# Autodesk Inventor assembly: Gantry Assembly
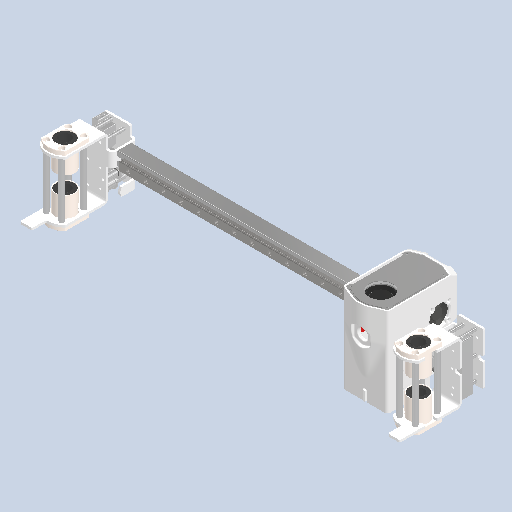
[picture p0: Inventor's stored thumbnail of the model, 512x512]
Saved by Autodesk Inventor 2024 (Build 280153000, 153)
## iProperties
Created: 2024-12-26
Part Number: Gantry Assembly
Document SubType Name: Assembly
Designer: Ishaan
Author: Ishaan
## Documents named in this file (15)
- E:\Projects\Axiom--IDEX-3D-Printer\CAD\04 - Gantry\Gantry Assembly.iam
- E:\Projects\Axiom--IDEX-3D-Printer\CAD\04 - Gantry\Left Gantry Guide.ipt
- E:\Projects\Axiom--IDEX-3D-Printer\CAD\00 - COTS Components\LMH16UU\LMH16UUx37\LMH16UUx37.ipt
- E:\Projects\Axiom--IDEX-3D-Printer\CAD\00 - COTS Components\Hardware\M3 30mm Standoff.ipt
- E:\Projects\Axiom--IDEX-3D-Printer\CAD\04 - Gantry\Right Gantry Guide.ipt
- E:\Projects\Axiom--IDEX-3D-Printer\CAD\04 - Gantry\Gantry Belt Clamp.ipt
- E:\Projects\Axiom--IDEX-3D-Printer\CAD\04 - Gantry\Gantry Belt Retainer.ipt
- E:\Projects\Axiom--IDEX-3D-Printer\CAD\00 - COTS Components\10mm 20T GT2 Idler Pulley 5mm Bore\10mm 20T GT2 Idler Pulley 5mm Bore.ipt
- E:\Projects\Axiom--IDEX-3D-Printer\CAD\00 - COTS Components\10mm Smooth Idler Pulley 5mm Bore\10mm 20T Smooth Idler Pulley 5mm Bore.ipt
- E:\Projects\Axiom--IDEX-3D-Printer\CAD\00 - COTS Components\Hardware\M5 Shim 0p5mm.ipt
- E:\Projects\Axiom--IDEX-3D-Printer\CAD\00 - COTS Components\Hardware\M5 Spacer 15mm.ipt
- E:\Projects\Axiom--IDEX-3D-Printer\CAD\00 - COTS Components\MGNR12 Rail\MGNR12R475HM.ipt
- E:\Projects\Axiom--IDEX-3D-Printer\CAD\05 - Printhead\Printhead Assembly.iam
- E:\Projects\Axiom--IDEX-3D-Printer\CAD\00 - COTS Components\Hardware\M4 80mm Standoff.ipt
- E:\Projects\Axiom--IDEX-3D-Printer\CAD\00 - COTS Components\2020 Gantry Extrusion\HFSH5-2020-446.ipt
## Components (57 placed, 14 different names)
1. Left Gantry Guide:1 — Insert:1, Insert:2, Insert:3, Insert:4, Insert:9, Insert:10, Insert:11, Insert:12, Insert:13, Insert:14, Insert:15, Insert:34, Insert:35, Insert:56, Insert:57, Insert:58, Insert:65, Insert:66, Insert:67
2. Right Gantry Guide:1 — Insert:17, Insert:18, Insert:19, Insert:20, Insert:25, Insert:26, Insert:27, Insert:28, Insert:29, Insert:30, Insert:31, Insert:48, Insert:49, Insert:52, Insert:54, Insert:62, Insert:63, Insert:64
3. HFSH5-2020-446:1
4. LMH16UUx37:1 — Insert:1, Insert:2
5. LMH16UUx37:2 — Insert:3, Insert:4
6. LMH16UUx37:3 — Insert:19, Insert:20
7. LMH16UUx37:4 — Insert:17, Insert:18
8. Gantry Belt Clamp:1 — Insert:36, Insert:37, Insert:38, Insert:39
9. Gantry Belt Retainer:1 — Insert:40, Insert:41
10. Gantry Belt Clamp:2 — Insert:38, Insert:39, Insert:40, Insert:41
11. Gantry Belt Retainer:2 — Insert:34, Insert:35, Insert:36, Insert:37
12. Gantry Belt Clamp:3
13. Gantry Belt Retainer:3
14. Gantry Belt Clamp:4
15. Gantry Belt Retainer:4 — Insert:48, Insert:49
16. 10mm 20T GT2 Idler Pulley 5mm Bore:1 — Insert:55
17. 10mm 20T GT2 Idler Pulley 5mm Bore:2 — Insert:61
18. 10mm 20T Smooth Idler Pulley 5mm Bore:1 — Insert:60
19. 10mm 20T Smooth Idler Pulley 5mm Bore:2 — Insert:59
20. 10mm 20T Smooth Idler Pulley 5mm Bore:3 — Insert:51
21. 10mm 20T Smooth Idler Pulley 5mm Bore:4 — Insert:53
22. M5 Spacer 15mm:1 — Insert:64
23. M5 Spacer 15mm:2 — Insert:63
24. M5 Spacer 15mm:3 — Insert:62
25. M5 Spacer 15mm:4 — Insert:67
26. M5 Spacer 15mm:5 — Insert:66
27. M5 Spacer 15mm:6 — Insert:65
28. MGNR12R475HM:1 — Mate:5
29. Printhead Assembly:1 [sub-assembly] — Mate:5
30. M5 Shim 0p5mm:1 — Insert:50, Insert:51
31. M5 Shim 0p5mm:2 — Insert:54, Insert:55
32. M5 Shim 0p5mm:3 — Insert:52, Insert:53
33. M5 Shim 0p5mm:4 — Insert:58, Insert:59
34. M5 Shim 0p5mm:5 — Insert:56, Insert:60
35. M5 Shim 0p5mm:6 — Insert:57, Insert:61
36. M3 30mm Standoff:8 — Insert:25
37. M3 30mm Standoff:9 — Insert:27
38. M3 30mm Standoff:10 — Insert:26
39. M3 30mm Standoff:11 — Insert:29
40. M3 30mm Standoff:12 — Insert:30
41. M3 30mm Standoff:13 — Insert:31
42. M3 30mm Standoff:14 — Insert:28, Insert:50
43. M4 80mm Standoff:1
44. M4 80mm Standoff:2
45. M4 80mm Standoff:3
46. M4 80mm Standoff:4
47. M4 80mm Standoff:5
48. M4 80mm Standoff:6
49. M4 80mm Standoff:7
50. M4 80mm Standoff:8
51. M3 30mm Standoff:1 — Insert:10
52. M3 30mm Standoff:2 — Insert:11
53. M3 30mm Standoff:3 — Insert:12
54. M3 30mm Standoff:4 — Insert:13
55. M3 30mm Standoff:5 — Insert:14
56. M3 30mm Standoff:6 — Insert:15
57. M3 30mm Standoff:7 — Insert:9
## Relationships (73: Insert 66, Mate 5, Angle 2)
- Insert:1: Left Gantry Guide:1 ↔ LMH16UUx37:1
- Insert:2: Left Gantry Guide:1 ↔ LMH16UUx37:1
- Insert:3: Left Gantry Guide:1 ↔ LMH16UUx37:2
- Insert:4: Left Gantry Guide:1 ↔ LMH16UUx37:2
- [Insert]: Left Gantry Guide:1 ↔ M4 80mm Standoff:8
- [Insert]: Left Gantry Guide:1 ↔ M4 80mm Standoff:7
- [Insert]: Left Gantry Guide:1 ↔ M4 80mm Standoff:6
- [Insert]: Left Gantry Guide:1 ↔ M4 80mm Standoff:5
- Insert:9: Left Gantry Guide:1 ↔ M3 30mm Standoff:7
- Insert:10: Left Gantry Guide:1 ↔ M3 30mm Standoff:1
- Insert:11: Left Gantry Guide:1 ↔ M3 30mm Standoff:2
- Insert:12: Left Gantry Guide:1 ↔ M3 30mm Standoff:3
- Insert:13: Left Gantry Guide:1 ↔ M3 30mm Standoff:4
- Insert:14: Left Gantry Guide:1 ↔ M3 30mm Standoff:5
- Insert:15: Left Gantry Guide:1 ↔ M3 30mm Standoff:6
- Insert:17: Right Gantry Guide:1 ↔ LMH16UUx37:4
- Insert:18: Right Gantry Guide:1 ↔ LMH16UUx37:4
- Insert:19: Right Gantry Guide:1 ↔ LMH16UUx37:3
- Insert:20: Right Gantry Guide:1 ↔ LMH16UUx37:3
- [Insert]: Right Gantry Guide:1 ↔ M4 80mm Standoff:1
- [Insert]: Right Gantry Guide:1 ↔ M4 80mm Standoff:2
- [Insert]: Right Gantry Guide:1 ↔ M4 80mm Standoff:3
- [Insert]: Right Gantry Guide:1 ↔ M4 80mm Standoff:4
- Insert:25: Right Gantry Guide:1 ↔ M3 30mm Standoff:8
- Insert:26: Right Gantry Guide:1 ↔ M3 30mm Standoff:10
- Insert:27: Right Gantry Guide:1 ↔ M3 30mm Standoff:9
- Insert:28: Right Gantry Guide:1 ↔ M3 30mm Standoff:14
- Insert:29: Right Gantry Guide:1 ↔ M3 30mm Standoff:11
- Insert:30: Right Gantry Guide:1 ↔ M3 30mm Standoff:12
- Insert:31: Right Gantry Guide:1 ↔ M3 30mm Standoff:13
- [Insert]: Left Gantry Guide:1 ↔ HFSH5-2020-446:1
- [Angle] (0 deg): Left Gantry Guide:1 ↔ HFSH5-2020-446:1
- [Insert]: Right Gantry Guide:1 ↔ HFSH5-2020-446:1
- [Angle] (0 deg): Right Gantry Guide:1 ↔ HFSH5-2020-446:1
- Insert:34: Left Gantry Guide:1 ↔ Gantry Belt Retainer:2
- Insert:35: Left Gantry Guide:1 ↔ Gantry Belt Retainer:2
- Insert:36: Gantry Belt Clamp:1 ↔ Gantry Belt Retainer:2
- Insert:37: Gantry Belt Clamp:1 ↔ Gantry Belt Retainer:2
- Insert:38: Gantry Belt Clamp:1 ↔ Gantry Belt Clamp:2
- Insert:39: Gantry Belt Clamp:1 ↔ Gantry Belt Clamp:2
- Insert:40: Gantry Belt Retainer:1 ↔ Gantry Belt Clamp:2
- Insert:41: Gantry Belt Retainer:1 ↔ Gantry Belt Clamp:2
- [Insert]: Gantry Belt Clamp:3 ↔ Gantry Belt Retainer:4
- [Insert]: Gantry Belt Clamp:3 ↔ Gantry Belt Retainer:4
- [Insert]: Gantry Belt Clamp:3 ↔ Gantry Belt Clamp:4
- [Insert]: Gantry Belt Clamp:3 ↔ Gantry Belt Clamp:4
- [Insert]: Gantry Belt Retainer:3 ↔ Gantry Belt Clamp:4
- [Insert]: Gantry Belt Retainer:3 ↔ Gantry Belt Clamp:4
- Insert:48: Right Gantry Guide:1 ↔ Gantry Belt Retainer:4
- Insert:49: Right Gantry Guide:1 ↔ Gantry Belt Retainer:4
- Insert:50: M5 Shim 0p5mm:1 ↔ M3 30mm Standoff:14
- Insert:51: 10mm 20T Smooth Idler Pulley 5mm Bore:3 ↔ M5 Shim 0p5mm:1
- Insert:52: Right Gantry Guide:1 ↔ M5 Shim 0p5mm:3
- Insert:53: 10mm 20T Smooth Idler Pulley 5mm Bore:4 ↔ M5 Shim 0p5mm:3
- Insert:54: Right Gantry Guide:1 ↔ M5 Shim 0p5mm:2
- Insert:55: 10mm 20T GT2 Idler Pulley 5mm Bore:1 ↔ M5 Shim 0p5mm:2
- Insert:56: Left Gantry Guide:1 ↔ M5 Shim 0p5mm:5
- Insert:57: Left Gantry Guide:1 ↔ M5 Shim 0p5mm:6
- Insert:58: Left Gantry Guide:1 ↔ M5 Shim 0p5mm:4
- Insert:59: 10mm 20T Smooth Idler Pulley 5mm Bore:2 ↔ M5 Shim 0p5mm:4
- Insert:60: 10mm 20T Smooth Idler Pulley 5mm Bore:1 ↔ M5 Shim 0p5mm:5
- Insert:61: 10mm 20T GT2 Idler Pulley 5mm Bore:2 ↔ M5 Shim 0p5mm:6
- Insert:62: Right Gantry Guide:1 ↔ M5 Spacer 15mm:3
- Insert:63: Right Gantry Guide:1 ↔ M5 Spacer 15mm:2
- Insert:64: Right Gantry Guide:1 ↔ M5 Spacer 15mm:1
- Insert:65: Left Gantry Guide:1 ↔ M5 Spacer 15mm:6
- Insert:66: Left Gantry Guide:1 ↔ M5 Spacer 15mm:5
- Insert:67: Left Gantry Guide:1 ↔ M5 Spacer 15mm:4
- [Mate]: HFSH5-2020-446:1 ↔ MGNR12R475HM:1
- [Mate]: HFSH5-2020-446:1 ↔ MGNR12R475HM:1
- [Mate]: HFSH5-2020-446:1 ↔ MGNR12R475HM:1
- [Mate] (13 mm): HFSH5-2020-446:1 ↔ Printhead Assembly:1
- Mate:5: MGNR12R475HM:1 ↔ Printhead Assembly:1
## Named parameters: d45_d39 = 0 mm, d46_d40 = 0 mm, d47_d41 = 0 mm, d48_d42 = 0 mm, d49_d43 = 0 mm, d50_d44 = 0 mm
